# Autodesk Inventor assembly: neopixel-minipcb
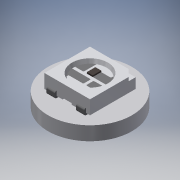
[picture p0: Inventor's stored thumbnail of the model, 180x180]
Saved by Autodesk Inventor 2018 (Build 220112000, 112)
## iProperties
Created: 2018-04-07
Part Number: neopixel-minipcb
Document SubType Name: Assembly
Designer: Raghava
Author: Raghava
## iProperties of the stored document ws2812-led.ipt
Created: 2014-08-01
Part Number: ws2812-led
Material: Generic
Document SubType Name: Modeling
Designer: Raghava
Density: 1 g/cm^3
Appearance: Default
Sending System: SIEMENS PLM Software NX 9.0
Preprocessor: ST-DEVELOPER v15
Title: WS2812_RGB_LED_updated.stp
## Documents named in this file (5)
- **C:\Users\Raghava\Desktop\scracktrackball\neopixel-minipcb.iam*LocalDocs*xBdwmfjzaAo2jescgMbje142eAf*ws2812-led.ipt
- C:\Users\Raghava\Desktop\iot-ball\cad\neopixel-minipcb.iam
- C:\Users\Raghava\Desktop\iot-ball\cad\small-pcb.ipt
- **C:\Users\Raghava\Desktop\iot-ball\cad\neopixel-minipcb.iam*LocalDocs*xBdwmfjzaAo2jescgMbje142eAf*ws2812-led.ipt
- C:\Users\Raghava\Desktop\iot-ball\cad\components\ws2812-led.stp
## Components (2 placed, 2 different names)
1. small-pcb:1 — Rigid:1
2. ws2812-led:1 — Rigid:1
## Relationships (1: WeldJoint 1)
- Rigid:1 [WeldJoint] (0.2 mm): small-pcb:1 ↔ ws2812-led:1
